# Autodesk Inventor assembly: CNC-Z-axis- ASSEMBLY
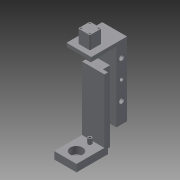
[picture p0: Inventor's stored thumbnail of the model, 180x180]
Saved by Autodesk Inventor 2015 (Build 190159000, 159)
## iProperties
Created: 2015-03-24
Part Number: CNC-Z-axis- ASSEMBLY
Document SubType Name: Assembly
Designer: Bangladesh
Author: Bangladesh
## Documents named in this file (8)
- C:\Users\Alvi\Documents\CNC design files\Assemblies\CNC-Z-axis- ASSEMBLY.iam
- C:\Users\Alvi\Documents\CNC design files\CNC-Z-axis- linear drawer slider.ipt
- C:\Users\Alvi\Documents\CNC design files\CNC-Y-axis- moving side to side plateform.ipt
- C:\Users\Alvi\Documents\CNC design files\CNC-Z-axis - backplate.ipt
- C:\Users\Alvi\Documents\CNC design files\CNC-Z-axis- dremel mount.ipt
- C:\Users\Alvi\Documents\CNC design files\CNC- Hexagonal Bit.ipt
- C:\Users\Alvi\Documents\CNC design files\CNC-Z-axis- top plate.ipt
- C:\Users\Alvi\Documents\CNC design files\CNC- Stepper Motor.ipt
## Components (8 placed, 7 different names)
1. CNC-Y-axis- moving side to side plateform:1 — Mate:1, Mate:2, Mate:10, Mate:11, Mate:14, Mate:15
2. CNC-Z-axis- linear drawer slider:1 — Mate:1, Mate:2, Mate:3, Flush:1, Mate:4
3. CNC-Z-axis - backplate:1 — Mate:3, Flush:1, Mate:4, Mate:5, Mate:6
4. CNC-Z-axis- dremel mount:1 — Mate:5, Mate:6, Mate:7, Mate:8, Mate:9
5. CNC- Hexagonal Bit:1 — Mate:7, Mate:8, Mate:9
6. CNC-Z-axis- top plate:1 — Mate:10, Mate:11, Mate:12, Mate:13
7. CNC- Stepper Motor:1 — Mate:12, Mate:13
8. CNC- Hexagonal Bit:2 — Mate:14, Mate:15
## Relationships (16: Mate 15, Flush 1)
- Mate:1 (22.86 mm): CNC-Y-axis- moving side to side plateform:1 ↔ CNC-Z-axis- linear drawer slider:1
- Mate:2 (68.7 mm): CNC-Y-axis- moving side to side plateform:1 ↔ CNC-Z-axis- linear drawer slider:1
- Mate:3: CNC-Z-axis- linear drawer slider:1 ↔ CNC-Z-axis - backplate:1
- Flush:1 (-18.4 mm): CNC-Z-axis- linear drawer slider:1 ↔ CNC-Z-axis - backplate:1
- Mate:4: CNC-Z-axis- linear drawer slider:1 ↔ CNC-Z-axis - backplate:1
- Mate:5: CNC-Z-axis - backplate:1 ↔ CNC-Z-axis- dremel mount:1
- Mate:6: CNC-Z-axis - backplate:1 ↔ CNC-Z-axis- dremel mount:1
- Mate:7: CNC-Z-axis- dremel mount:1 ↔ CNC- Hexagonal Bit:1
- Mate:8: CNC-Z-axis- dremel mount:1 ↔ CNC- Hexagonal Bit:1
- Mate:9: CNC-Z-axis- dremel mount:1 ↔ CNC- Hexagonal Bit:1
- Mate:10: CNC-Y-axis- moving side to side plateform:1 ↔ CNC-Z-axis- top plate:1
- Mate:11: CNC-Y-axis- moving side to side plateform:1 ↔ CNC-Z-axis- top plate:1
- Mate:12: CNC-Z-axis- top plate:1 ↔ CNC- Stepper Motor:1
- Mate:13: CNC-Z-axis- top plate:1 ↔ CNC- Stepper Motor:1
- Mate:14: CNC-Y-axis- moving side to side plateform:1 ↔ CNC- Hexagonal Bit:2
- Mate:15: CNC-Y-axis- moving side to side plateform:1 ↔ CNC- Hexagonal Bit:2
